# Autodesk Inventor assembly: Electronics_Assy
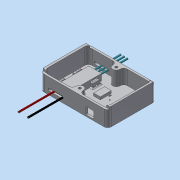
[picture p0: Inventor's stored thumbnail of the model, 180x180]
Saved by Autodesk Inventor 2015 SP1 (Build 190203100, 203)
## iProperties
Created: 2015-06-23
Part Number: Electronics_Assy
Document SubType Name: Assembly
Designer: YOUR_NAME_HERE
Author: YOUR_NAME_HERE
## Documents named in this file (3)
- C:\Users\Rahul\Electric Skateboard\Electric Skateboard CAD\Electronics_Assy.iam
- C:\Users\Rahul\Electric Skateboard\Electric Skateboard CAD\ControlElectronicsBox.ipt
- C:\Users\Rahul\Electric Skateboard\Electric Skateboard CAD\Turnigy_ESC.ipt
## Components (2 placed, 2 different names)
1. ControlElectronicsBox:1 — Flush:1, Mate:1
2. Turnigy_ESC:1 — Flush:1, Mate:1
## Relationships (2: Flush 1, Mate 1)
- Flush:1: ControlElectronicsBox:1 ↔ Turnigy_ESC:1
- Mate:1: ControlElectronicsBox:1 ↔ Turnigy_ESC:1
